# Autodesk Inventor assembly: Gear HS 36 tooth
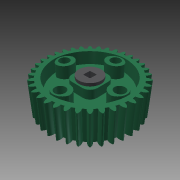
[picture p0: Inventor's stored thumbnail of the model, 180x180]
Saved by Autodesk Inventor 2015 (Build 190159000, 159)
## iProperties
Created: 2014-04-22
Part Number: Gear HS 36 tooth
Document SubType Name: Assembly
Designer: Christopher Vodney
Author: Christopher Vodney
## Documents named in this file (3)
- F:\VEX CAD Library\Motion\Gear HS 36 tooth.iam
- F:\VEX CAD Library\Motion\Gear HS 36 tooth.ipt
- F:\VEX CAD Library\Motion\Insert HS Metal.ipt
## Components (3 placed, 2 different names)
1. Gear HS 36 tooth:1 — Mate:5, Mate:6, Angle:3, Mate:7, Mate:8, Angle:4
2. Insert HS Metal:1 — Mate:7, Mate:8, Angle:4
3. Insert HS Metal:2 — Mate:5, Mate:6, Angle:3
## Relationships (6: Mate 4, Angle 2)
- Mate:5: Gear HS 36 tooth:1 ↔ Insert HS Metal:2
- Mate:6: Gear HS 36 tooth:1 ↔ Insert HS Metal:2
- Angle:3 (0 deg): Gear HS 36 tooth:1 ↔ Insert HS Metal:2
- Mate:7: Gear HS 36 tooth:1 ↔ Insert HS Metal:1
- Mate:8: Gear HS 36 tooth:1 ↔ Insert HS Metal:1
- Angle:4 (0 deg): Gear HS 36 tooth:1 ↔ Insert HS Metal:1
